# Autodesk Inventor assembly: MonteCarloM1.1
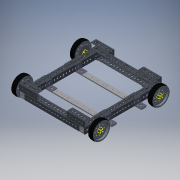
[picture p0: Inventor's stored thumbnail of the model, 180x180]
Saved by Autodesk Inventor 2016 (Build 200138000, 138)
## iProperties
Created: 2015-09-04
Part Number: MonteCarloM1.1
Document SubType Name: Assembly
Designer: Tim
Author: Tim
## Documents named in this file (9)
- C:\Users\phi\Documents\GitHub\phi_robotics\3d-models\FTC_Tetrix_KOP_Block_Party\Tim Bloot Designs\MonteCarloM1.1.iam
- C:\Users\phi\Documents\GitHub\phi_robotics\3d-models\FTC_Tetrix_KOP_Block_Party\Tetrix_Kit_FTC\Autodesk Inventor Files\tetrix_c_channel-5.ipt
- C:\Users\phi\Documents\GitHub\phi_robotics\3d-models\FTC_Tetrix_KOP_Block_Party\Tetrix_Kit_FTC\Autodesk Inventor Files\tetrix_c_channel-4.ipt
- C:\Users\phi\Documents\GitHub\phi_robotics\3d-models\FTC_Tetrix_KOP_Block_Party\Tetrix_Kit_FTC\Autodesk Inventor Files\tetrix_c_channel-2.ipt
- C:\Users\phi\Documents\GitHub\phi_robotics\3d-models\FTC_Tetrix_KOP_Block_Party\Tetrix_Kit_FTC\Autodesk Inventor Files\tetrix_c_channel-round.ipt
- C:\Users\phi\Documents\GitHub\phi_robotics\3d-models\FTC_Tetrix_KOP_Block_Party\Tetrix_Kit_FTC\Autodesk Inventor Files\tetrix_inside_corner_bracket.ipt
- C:\Users\phi\Documents\GitHub\phi_robotics\3d-models\FTC_Tetrix_KOP_Block_Party\WheelNChainGear.iam
- C:\Users\phi\Documents\GitHub\phi_robotics\3d-models\FTC_Tetrix_KOP_Block_Party\Tetrix_Kit_FTC\Autodesk Inventor Files\tetrix_bushing.ipt
- C:\Users\phi\Documents\GitHub\phi_robotics\3d-models\FTC_Tetrix_KOP_Block_Party\Tim Bloot Designs\MCbeam.ipt
## Components (34 placed, 8 different names)
1. tetrix_c_channel-5:1 — Rigid:1, Rigid:4, Rigid:9, Rigid:12, Rigid:15, Rigid:16, Rigid:19, Rigid:20, Rotational:1, Rotational:2, Rotational:7, Rotational:8
2. tetrix_c_channel-5:2 — Rigid:2, Rigid:3, Rigid:10, Rigid:11, Rigid:13, Rigid:14, Rigid:17, Rigid:18, Rotational:3, Rotational:4, Rotational:5, Rotational:6
3. tetrix_c_channel-4:1 — Rigid:7, Rigid:8
4. tetrix_c_channel-4:2 — Rigid:5, Rigid:6
5. tetrix_c_channel-2:1 — Rigid:1, Rigid:7
6. tetrix_c_channel-2:2 — Rigid:2, Rigid:8
7. tetrix_c_channel-2:3 — Rigid:3, Rigid:6
8. tetrix_c_channel-2:4 — Rigid:4, Rigid:5
9. tetrix_c_channel-round:1 — Rigid:9
10. tetrix_c_channel-round:2 — Rigid:10
11. tetrix_c_channel-round:3 — Rigid:12
12. tetrix_c_channel-round:4 — Rigid:11
13. tetrix_inside_corner_bracket:1 — Rigid:19
14. tetrix_inside_corner_bracket:2 — Rigid:20
15. tetrix_inside_corner_bracket:3 — Rigid:14
16. tetrix_inside_corner_bracket:4 — Rigid:13
17. tetrix_inside_corner_bracket:5 — Rigid:16, Rigid:22
18. tetrix_inside_corner_bracket:6 — Rigid:15, Rigid:21
19. tetrix_inside_corner_bracket:7 — Rigid:18, Rigid:24
20. tetrix_inside_corner_bracket:8 — Rigid:17, Rigid:23
21. WheelNChainGear:1 [sub-assembly] — Rotational:12
22. WheelNChainGear:2 [sub-assembly] — Rotational:11
23. WheelNChainGear:3 [sub-assembly] — Rotational:10
24. WheelNChainGear:4 [sub-assembly] — Rotational:9
25. tetrix_bushing:1 — Rotational:3, Rotational:9
26. tetrix_bushing:2 — Rotational:4, Rotational:10
27. tetrix_bushing:3 — Rotational:1
28. tetrix_bushing:4 — Rotational:2
29. tetrix_bushing:5 — Rotational:7, Rotational:11
30. tetrix_bushing:6 — Rotational:8, Rotational:12
31. tetrix_bushing:7 — Rotational:6
32. tetrix_bushing:8 — Rotational:5
33. MCbeam:1 — Rigid:21, Rigid:23
34. MCbeam:3 — Rigid:22, Rigid:24
## Relationships (36: WeldJoint 24, RevoluteJoint 12)
- Rigid:1 [WeldJoint]: tetrix_c_channel-5:1 ↔ tetrix_c_channel-2:1
- Rigid:2 [WeldJoint]: tetrix_c_channel-5:2 ↔ tetrix_c_channel-2:2
- Rigid:3 [WeldJoint]: tetrix_c_channel-5:2 ↔ tetrix_c_channel-2:3
- Rigid:4 [WeldJoint]: tetrix_c_channel-5:1 ↔ tetrix_c_channel-2:4
- Rigid:5 [WeldJoint]: tetrix_c_channel-4:2 ↔ tetrix_c_channel-2:4
- Rigid:6 [WeldJoint]: tetrix_c_channel-4:2 ↔ tetrix_c_channel-2:3
- Rigid:7 [WeldJoint]: tetrix_c_channel-4:1 ↔ tetrix_c_channel-2:1
- Rigid:8 [WeldJoint]: tetrix_c_channel-4:1 ↔ tetrix_c_channel-2:2
- Rigid:9 [WeldJoint]: tetrix_c_channel-5:1 ↔ tetrix_c_channel-round:1
- Rigid:10 [WeldJoint]: tetrix_c_channel-5:2 ↔ tetrix_c_channel-round:2
- Rigid:11 [WeldJoint]: tetrix_c_channel-5:2 ↔ tetrix_c_channel-round:4
- Rigid:12 [WeldJoint]: tetrix_c_channel-5:1 ↔ tetrix_c_channel-round:3
- Rigid:13 [WeldJoint]: tetrix_c_channel-5:2 ↔ tetrix_inside_corner_bracket:4
- Rigid:14 [WeldJoint]: tetrix_c_channel-5:2 ↔ tetrix_inside_corner_bracket:3
- Rigid:15 [WeldJoint]: tetrix_c_channel-5:1 ↔ tetrix_inside_corner_bracket:6
- Rigid:16 [WeldJoint]: tetrix_c_channel-5:1 ↔ tetrix_inside_corner_bracket:5
- Rigid:17 [WeldJoint]: tetrix_c_channel-5:2 ↔ tetrix_inside_corner_bracket:8
- Rigid:18 [WeldJoint]: tetrix_c_channel-5:2 ↔ tetrix_inside_corner_bracket:7
- Rigid:19 [WeldJoint]: tetrix_c_channel-5:1 ↔ tetrix_inside_corner_bracket:1
- Rigid:20 [WeldJoint]: tetrix_c_channel-5:1 ↔ tetrix_inside_corner_bracket:2
- Rotational:1 [RevoluteJoint]: tetrix_c_channel-5:1 ↔ tetrix_bushing:3
- Rotational:2 [RevoluteJoint]: tetrix_c_channel-5:1 ↔ tetrix_bushing:4
- Rotational:3 [RevoluteJoint]: tetrix_c_channel-5:2 ↔ tetrix_bushing:1
- Rotational:4 [RevoluteJoint]: tetrix_c_channel-5:2 ↔ tetrix_bushing:2
- Rotational:5 [RevoluteJoint]: tetrix_c_channel-5:2 ↔ tetrix_bushing:8
- Rotational:6 [RevoluteJoint]: tetrix_c_channel-5:2 ↔ tetrix_bushing:7
- Rotational:7 [RevoluteJoint]: tetrix_c_channel-5:1 ↔ tetrix_bushing:5
- Rotational:8 [RevoluteJoint]: tetrix_c_channel-5:1 ↔ tetrix_bushing:6
- Rotational:9 [RevoluteJoint] (-20 mm): WheelNChainGear:4 ↔ tetrix_bushing:1
- Rotational:10 [RevoluteJoint] (-25 mm): WheelNChainGear:3 ↔ tetrix_bushing:2
- Rotational:11 [RevoluteJoint] (-25 mm): WheelNChainGear:2 ↔ tetrix_bushing:5
- Rotational:12 [RevoluteJoint] (-25 mm): WheelNChainGear:1 ↔ tetrix_bushing:6
- Rigid:21 [WeldJoint]: tetrix_inside_corner_bracket:6 ↔ MCbeam:1
- Rigid:22 [WeldJoint]: tetrix_inside_corner_bracket:5 ↔ MCbeam:3
- Rigid:23 [WeldJoint]: tetrix_inside_corner_bracket:8 ↔ MCbeam:1
- Rigid:24 [WeldJoint]: tetrix_inside_corner_bracket:7 ↔ MCbeam:3
